# Autodesk Inventor assembly: V2 Output-90Deg
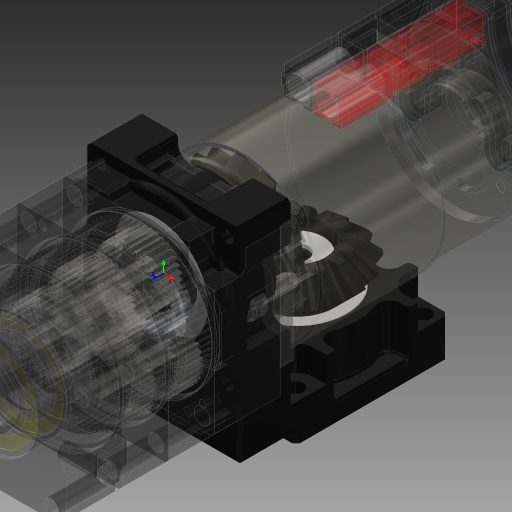
[picture p0: Inventor's stored thumbnail of the model, 512x512]
Saved by Autodesk Inventor 2023 (Build 270158000, 158)
## iProperties
Created: 2018-08-19
Part Number: V2 Output-90Deg
Document SubType Name: Assembly
Mass: 68.0389 g
Surface Area: 377.272 cm^2
Volume: 60.8381 cm^3
Density: 1.11836 g/cm^3
## Documents named in this file (3)
- C:\Users\Cal\Desktop\Robotics\Design\Collaborative\Collaborative Parts Library\General Gearboxes\Planetaries\Versaplanetary\V2 Stages\V2 Output Stage\V2 Output Stage 90 deg.iam
- C:\Users\Cal\Desktop\Robotics\Design\Collaborative\Collaborative Parts Library\General Gearboxes\Planetaries\Versaplanetary\VP 90 deg.ipt
- C:\Users\Cal\Desktop\Robotics\Design\Collaborative\Collaborative Parts Library\General Gearboxes\Planetaries\Versaplanetary\V2 Stages\V2 Output Stage.iam
## Components (1 placed, 1 different names)
1. VP 90 deg:1 — Flush:8, Mate:5, Angle:7
## Relationships (3: Flush 1, Mate 1, Angle 1)
- Flush:8: VP 90 deg:1
- Mate:5: VP 90 deg:1
- Angle:7 (0 deg): VP 90 deg:1
